# Autodesk Inventor assembly: Super Gantry
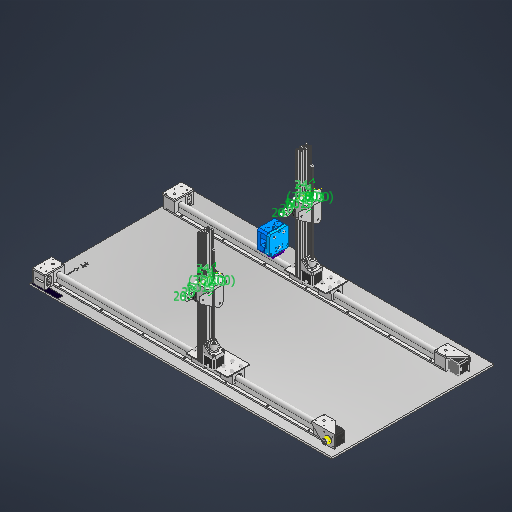
[picture p0: Inventor's stored thumbnail of the model, 512x512]
Saved by Autodesk Inventor 2025.1 (Build 291241000, 241)
## iProperties
Created: 2025-01-22
Part Number: Super Gantry
Document SubType Name: Assembly
Designer: jerem
Author: jerem
## Documents named in this file (5)
- C:\Users\jerem\Documents\GitHub\Perovskite-Automated-Synthesis-System\CAD\Gantry\Super Gantry.iam
- C:\Users\jerem\Documents\GitHub\Perovskite-Automated-Synthesis-System\CAD\Gantry\X Axis.iam
- C:\Users\jerem\Documents\GitHub\Perovskite-Automated-Synthesis-System\CAD\Gantry\Z Axis.iam
- C:\Users\jerem\Documents\GitHub\Perovskite-Automated-Synthesis-System\CAD\Toolhead\Toolhead.iam
- C:\Users\jerem\Documents\GitHub\Perovskite-Automated-Synthesis-System\CAD\Camera\Camera Assembly.iam
## Components (5 placed, 4 different names)
1. X Axis:1 [sub-assembly] — Mate:1, Mate:2, Mate:3, Mate:4, Mate:5, Mate:6
2. Z Axis:1 [sub-assembly] — Mate:4, Mate:5, Mate:6
3. Z Axis:2 [sub-assembly] — Mate:1, Mate:2, Mate:3
4. Toolhead:1 [sub-assembly] — Mate:8, Mate:9, Mate:10
5. Camera Assembly:1 [sub-assembly] — Mate:8, Mate:9, Mate:10
## Relationships (9: Mate 9)
- Mate:1: X Axis:1 ↔ Z Axis:2
- Mate:2: X Axis:1 ↔ Z Axis:2
- Mate:3: X Axis:1 ↔ Z Axis:2
- Mate:4: X Axis:1 ↔ Z Axis:1
- Mate:5: X Axis:1 ↔ Z Axis:1
- Mate:6: X Axis:1 ↔ Z Axis:1
- Mate:8: Toolhead:1 ↔ Camera Assembly:1
- Mate:9: Toolhead:1 ↔ Camera Assembly:1
- Mate:10: Toolhead:1 ↔ Camera Assembly:1
